# Autodesk Inventor assembly: Piston Build Platform assy
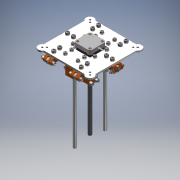
[picture p0: Inventor's stored thumbnail of the model, 180x180]
Saved by Autodesk Inventor 2018 (Build 220112000, 112)
## iProperties
Created: 2017-09-27
Part Number: Piston Build Platform assy
Document SubType Name: Assembly
Designer: Gabriel Smolnycki
Author: Gabriel Smolnycki
## Documents named in this file (11)
- H:\dev\planb\mechanics\V1INV\Subassemblies\Piston Build Platform assy.iam
- H:\dev\planb\mechanics\V1INV\Piston\Piston Build Frame.ipt
- H:\dev\planb\mechanics\V1INV\Subassemblies\Piston Wall Guide assy.iam
- H:\dev\planb\mechanics\V1INV\Hardware\M4 SS Washer.ipt
- H:\dev\planb\mechanics\V1INV\Hardware\M4 SS Locknut.ipt
- H:\dev\planb\mechanics\V1INV\Hardware\M4x25 SS SHCS.ipt
- H:\dev\planb\mechanics\V1INV\Subassemblies\Piston Motor Holder assy.iam
- H:\dev\planb\mechanics\V1INV\Hardware\M4x12 SS SHCS.ipt
- H:\dev\planb\mechanics\V1INV\Hardware\M4x30 SS Standoff FF (94868A183).ipt
- H:\dev\planb\mechanics\V1INV\Subassemblies\Piston Guide assy.iam
- H:\dev\planb\mechanics\V1INV\Hardware\M4x20 SS SHCS.ipt
## Components (118 placed, 10 different names)
1. Piston Build Frame:1 — Insert:1, Insert:2, Insert:3, Insert:4, Insert:5, Insert:6, Insert:7, Insert:8, Insert:9, Insert:10, Insert:11, Insert:12, Insert:13, Insert:14, Insert:15, Insert:16, Insert:17, Insert:18, Insert:19, Insert:20, Insert:21, Insert:22, Insert:23, Insert:24, Insert:61, Insert:62, Insert:63, Insert:64, Insert:65, Insert:66, Insert:67, Insert:68, Insert:91, Insert:92, Insert:93, Insert:94, Insert:95, Insert:96, Insert:97, Insert:98, Insert:99, Insert:100, Insert:101, Insert:102
2. Piston Wall Guide assy:1 [sub-assembly] — Insert:1, Insert:2, Insert:27, Insert:28
3. Piston Wall Guide assy:2 [sub-assembly] — Insert:3, Insert:4, Insert:25, Insert:26
4. Piston Wall Guide assy:3 [sub-assembly] — Insert:7, Insert:8, Insert:31, Insert:32
5. Piston Wall Guide assy:4 [sub-assembly] — Insert:5, Insert:6, Insert:29, Insert:30
6. Piston Wall Guide assy:5 [sub-assembly] — Insert:11, Insert:12, Insert:35, Insert:36
7. Piston Wall Guide assy:6 [sub-assembly] — Insert:9, Insert:10, Insert:33, Insert:34
8. M4x25 SS SHCS:1
9. M4x25 SS SHCS:2
10. M4x25 SS SHCS:3
11. M4x25 SS SHCS:4
12. M4x25 SS SHCS:5
13. M4x25 SS SHCS:6
14. M4x25 SS SHCS:7
15. M4x25 SS SHCS:8
16. M4x25 SS SHCS:9
17. M4x25 SS SHCS:10
18. M4x25 SS SHCS:11
19. M4x25 SS SHCS:12
20. M4 SS Washer:1 — Insert:14
21. M4 SS Washer:2 — Insert:16
22. M4 SS Washer:3 — Insert:21
23. M4 SS Washer:4 — Insert:22
24. M4 SS Washer:5 — Insert:13
25. M4 SS Washer:6 — Insert:17
26. M4 SS Washer:7 — Insert:20
27. M4 SS Washer:8 — Insert:36, Insert:48
28. M4 SS Washer:9 — Insert:15
29. M4 SS Washer:10 — Insert:18
30. M4 SS Washer:11 — Insert:19
31. M4 SS Washer:12 — Insert:23
32. M4 SS Washer:13 — Insert:32, Insert:44
33. M4 SS Washer:14 — Insert:31, Insert:43
34. M4 SS Washer:15 — Insert:30, Insert:39
35. M4 SS Washer:16 — Insert:29, Insert:40
36. M4 SS Washer:17 — Insert:35, Insert:47
37. M4 SS Washer:18 — Insert:34, Insert:46
38. M4 SS Washer:19 — Insert:33, Insert:45
39. M4 SS Washer:20 — Insert:28, Insert:42
40. M4 SS Washer:21 — Insert:24
41. M4 SS Washer:22 — Insert:27, Insert:41
42. M4 SS Washer:23 — Insert:26, Insert:38
43. M4 SS Washer:24 — Insert:25, Insert:37
44. M4 SS Locknut:1 — Insert:46
45. M4 SS Locknut:2 — Insert:45
46. M4 SS Locknut:3 — Insert:43
47. M4 SS Locknut:4 — Insert:41
48. M4 SS Locknut:5 — Insert:39
49. M4 SS Locknut:6 — Insert:37
50. M4 SS Locknut:7 — Insert:48
51. M4 SS Locknut:8 — Insert:47
52. M4 SS Locknut:9 — Insert:44
53. M4 SS Locknut:10 — Insert:42
54. M4 SS Locknut:11 — Insert:40
55. M4 SS Locknut:12 — Insert:38
56. Piston Motor Holder assy:1 [sub-assembly] — Insert:73, Insert:74, Insert:75, Insert:76, Insert:77, Insert:78, Insert:79, Insert:80
57. M4x12 SS SHCS:1
58. M4x12 SS SHCS:2
59. M4x12 SS SHCS:3
60. M4x12 SS SHCS:4
61. M4 SS Washer:25 — Insert:64
62. M4 SS Washer:26 — Insert:63
63. M4 SS Washer:27 — Insert:62
64. M4 SS Washer:28 — Insert:61
65. M4 SS Washer:29 — Insert:66, Insert:86
66. M4 SS Washer:30 — Insert:67, Insert:85
67. M4 SS Washer:31 — Insert:68, Insert:87
68. M4 SS Washer:32 — Insert:65, Insert:88
69. M4 SS Washer:33 — Insert:73, Insert:84
70. M4 SS Washer:34 — Insert:80, Insert:90
71. M4 SS Washer:35 — Insert:79
72. M4 SS Washer:36 — Insert:78, Insert:89
73. M4 SS Washer:37 — Insert:74, Insert:83
74. M4 SS Washer:38 — Insert:75, Insert:81
75. M4 SS Washer:39 — Insert:76, Insert:82
76. M4 SS Washer:40 — Insert:77
77. M4x12 SS SHCS:5 — Insert:81
78. M4x12 SS SHCS:6 — Insert:82
79. M4x12 SS SHCS:7 — Insert:84
80. M4x12 SS SHCS:8 — Insert:83
81. M4x30 SS Standoff FF (94868A183):1 — Insert:85, Insert:89
82. M4x30 SS Standoff FF (94868A183):2 — Insert:86
83. M4x30 SS Standoff FF (94868A183):3 — Insert:87
84. M4x30 SS Standoff FF (94868A183):4 — Insert:88, Insert:90
85. Piston Guide assy:1 [sub-assembly] — Insert:91, Insert:92, Insert:107, Insert:108, Insert:109, Insert:110
86. Piston Guide assy:2 [sub-assembly] — Insert:93, Insert:94, Insert:103, Insert:104, Insert:105, Insert:106
87. M4x20 SS SHCS:1
88. M4x20 SS SHCS:2
89. M4x20 SS SHCS:3
90. M4x20 SS SHCS:4
91. M4x20 SS SHCS:5
92. M4x20 SS SHCS:6
93. M4x20 SS SHCS:7
94. M4x20 SS SHCS:8
95. M4 SS Washer:41 — Insert:95
96. M4 SS Washer:42 — Insert:96
97. M4 SS Washer:43 — Insert:97
98. M4 SS Washer:44 — Insert:98
99. M4 SS Washer:45 — Insert:99
100. M4 SS Washer:46 — Insert:100
101. M4 SS Washer:47 — Insert:101
102. M4 SS Washer:48 — Insert:102
103. M4 SS Washer:49 — Insert:106, Insert:118
104. M4 SS Washer:50 — Insert:107, Insert:114
105. M4 SS Washer:51 — Insert:108, Insert:111
106. M4 SS Washer:52 — Insert:109, Insert:112
107. M4 SS Washer:53 — Insert:103, Insert:116
108. M4 SS Washer:54 — Insert:104, Insert:115
109. M4 SS Washer:55 — Insert:105, Insert:117
110. M4 SS Washer:56 — Insert:110, Insert:113
111. M4 SS Locknut:13 — Insert:111
112. M4 SS Locknut:14 — Insert:112
113. M4 SS Locknut:15 — Insert:113
114. M4 SS Locknut:16 — Insert:114
115. M4 SS Locknut:17 — Insert:115
116. M4 SS Locknut:18 — Insert:116
117. M4 SS Locknut:19 — Insert:117
118. M4 SS Locknut:20 — Insert:118
## Relationships (126: Insert 126)
- Insert:1: Piston Build Frame:1 ↔ Piston Wall Guide assy:1
- Insert:2: Piston Build Frame:1 ↔ Piston Wall Guide assy:1
- Insert:3: Piston Build Frame:1 ↔ Piston Wall Guide assy:2
- Insert:4: Piston Build Frame:1 ↔ Piston Wall Guide assy:2
- Insert:5: Piston Build Frame:1 ↔ Piston Wall Guide assy:4
- Insert:6: Piston Build Frame:1 ↔ Piston Wall Guide assy:4
- Insert:7: Piston Build Frame:1 ↔ Piston Wall Guide assy:3
- Insert:8: Piston Build Frame:1 ↔ Piston Wall Guide assy:3
- Insert:9: Piston Build Frame:1 ↔ Piston Wall Guide assy:6
- Insert:10: Piston Build Frame:1 ↔ Piston Wall Guide assy:6
- Insert:11: Piston Build Frame:1 ↔ Piston Wall Guide assy:5
- Insert:12: Piston Build Frame:1 ↔ Piston Wall Guide assy:5
- Insert:13: Piston Build Frame:1 ↔ M4 SS Washer:5
- Insert:14: Piston Build Frame:1 ↔ M4 SS Washer:1
- Insert:15: Piston Build Frame:1 ↔ M4 SS Washer:9
- Insert:16: Piston Build Frame:1 ↔ M4 SS Washer:2
- Insert:17: Piston Build Frame:1 ↔ M4 SS Washer:6
- Insert:18: Piston Build Frame:1 ↔ M4 SS Washer:10
- Insert:19: Piston Build Frame:1 ↔ M4 SS Washer:11
- Insert:20: Piston Build Frame:1 ↔ M4 SS Washer:7
- Insert:21: Piston Build Frame:1 ↔ M4 SS Washer:3
- Insert:22: Piston Build Frame:1 ↔ M4 SS Washer:4
- Insert:23: Piston Build Frame:1 ↔ M4 SS Washer:12
- Insert:24: Piston Build Frame:1 ↔ M4 SS Washer:21
- Insert:25: Piston Wall Guide assy:2 ↔ M4 SS Washer:24
- Insert:26: Piston Wall Guide assy:2 ↔ M4 SS Washer:23
- Insert:27: Piston Wall Guide assy:1 ↔ M4 SS Washer:22
- Insert:28: Piston Wall Guide assy:1 ↔ M4 SS Washer:20
- Insert:29: Piston Wall Guide assy:4 ↔ M4 SS Washer:16
- Insert:30: Piston Wall Guide assy:4 ↔ M4 SS Washer:15
- Insert:31: Piston Wall Guide assy:3 ↔ M4 SS Washer:14
- Insert:32: Piston Wall Guide assy:3 ↔ M4 SS Washer:13
- Insert:33: Piston Wall Guide assy:6 ↔ M4 SS Washer:19
- Insert:34: Piston Wall Guide assy:6 ↔ M4 SS Washer:18
- Insert:35: Piston Wall Guide assy:5 ↔ M4 SS Washer:17
- Insert:36: Piston Wall Guide assy:5 ↔ M4 SS Washer:8
- Insert:37: M4 SS Washer:24 ↔ M4 SS Locknut:6
- Insert:38: M4 SS Washer:23 ↔ M4 SS Locknut:12
- Insert:39: M4 SS Washer:15 ↔ M4 SS Locknut:5
- Insert:40: M4 SS Washer:16 ↔ M4 SS Locknut:11
- Insert:41: M4 SS Washer:22 ↔ M4 SS Locknut:4
- Insert:42: M4 SS Washer:20 ↔ M4 SS Locknut:10
- Insert:43: M4 SS Washer:14 ↔ M4 SS Locknut:3
- Insert:44: M4 SS Washer:13 ↔ M4 SS Locknut:9
- Insert:45: M4 SS Washer:19 ↔ M4 SS Locknut:2
- Insert:46: M4 SS Washer:18 ↔ M4 SS Locknut:1
- Insert:47: M4 SS Washer:17 ↔ M4 SS Locknut:8
- Insert:48: M4 SS Washer:8 ↔ M4 SS Locknut:7
- [Insert]: M4x25 SS SHCS:12 ↔ M4 SS Washer:9
- [Insert]: M4x25 SS SHCS:11 ↔ M4 SS Washer:2
- [Insert]: M4x25 SS SHCS:3 ↔ M4 SS Washer:6
- [Insert]: M4x25 SS SHCS:4 ↔ M4 SS Washer:10
- [Insert]: M4x25 SS SHCS:5 ↔ M4 SS Washer:7
- [Insert]: M4x25 SS SHCS:6 ↔ M4 SS Washer:11
- [Insert]: M4x25 SS SHCS:9 ↔ M4 SS Washer:5
- [Insert]: M4x25 SS SHCS:10 ↔ M4 SS Washer:1
- [Insert]: M4x25 SS SHCS:1 ↔ M4 SS Washer:12
- [Insert]: M4x25 SS SHCS:2 ↔ M4 SS Washer:21
- [Insert]: M4x25 SS SHCS:7 ↔ M4 SS Washer:3
- [Insert]: M4x25 SS SHCS:8 ↔ M4 SS Washer:4
- Insert:61: Piston Build Frame:1 ↔ M4 SS Washer:28
- Insert:62: Piston Build Frame:1 ↔ M4 SS Washer:27
- Insert:63: Piston Build Frame:1 ↔ M4 SS Washer:26
- Insert:64: Piston Build Frame:1 ↔ M4 SS Washer:25
- Insert:65: Piston Build Frame:1 ↔ M4 SS Washer:32
- Insert:66: Piston Build Frame:1 ↔ M4 SS Washer:29
- Insert:67: Piston Build Frame:1 ↔ M4 SS Washer:30
- Insert:68: Piston Build Frame:1 ↔ M4 SS Washer:31
- [Insert]: M4x12 SS SHCS:1 ↔ M4 SS Washer:27
- [Insert]: M4x12 SS SHCS:3 ↔ M4 SS Washer:28
- [Insert]: M4x12 SS SHCS:2 ↔ M4 SS Washer:25
- [Insert]: M4x12 SS SHCS:4 ↔ M4 SS Washer:26
- Insert:73: Piston Motor Holder assy:1 ↔ M4 SS Washer:33
- Insert:74: Piston Motor Holder assy:1 ↔ M4 SS Washer:37
- Insert:75: Piston Motor Holder assy:1 ↔ M4 SS Washer:38
- Insert:76: Piston Motor Holder assy:1 ↔ M4 SS Washer:39
- Insert:77: Piston Motor Holder assy:1 ↔ M4 SS Washer:40
- Insert:78: Piston Motor Holder assy:1 ↔ M4 SS Washer:36
- Insert:79: Piston Motor Holder assy:1 ↔ M4 SS Washer:35
- Insert:80: Piston Motor Holder assy:1 ↔ M4 SS Washer:34
- Insert:81: M4 SS Washer:38 ↔ M4x12 SS SHCS:5
- Insert:82: M4 SS Washer:39 ↔ M4x12 SS SHCS:6
- Insert:83: M4 SS Washer:37 ↔ M4x12 SS SHCS:8
- Insert:84: M4 SS Washer:33 ↔ M4x12 SS SHCS:7
- Insert:85: M4 SS Washer:30 ↔ M4x30 SS Standoff FF (94868A183):1
- Insert:86: M4 SS Washer:29 ↔ M4x30 SS Standoff FF (94868A183):2
- Insert:87: M4 SS Washer:31 ↔ M4x30 SS Standoff FF (94868A183):3
- Insert:88: M4 SS Washer:32 ↔ M4x30 SS Standoff FF (94868A183):4
- Insert:89: M4 SS Washer:36 ↔ M4x30 SS Standoff FF (94868A183):1
- Insert:90: M4 SS Washer:34 ↔ M4x30 SS Standoff FF (94868A183):4
- Insert:91: Piston Build Frame:1 ↔ Piston Guide assy:1
- Insert:92: Piston Build Frame:1 ↔ Piston Guide assy:1
- Insert:93: Piston Build Frame:1 ↔ Piston Guide assy:2
- Insert:94: Piston Build Frame:1 ↔ Piston Guide assy:2
- Insert:95: Piston Build Frame:1 ↔ M4 SS Washer:41
- Insert:96: Piston Build Frame:1 ↔ M4 SS Washer:42
- Insert:97: Piston Build Frame:1 ↔ M4 SS Washer:43
- Insert:98: Piston Build Frame:1 ↔ M4 SS Washer:44
- Insert:99: Piston Build Frame:1 ↔ M4 SS Washer:45
- Insert:100: Piston Build Frame:1 ↔ M4 SS Washer:46
- Insert:101: Piston Build Frame:1 ↔ M4 SS Washer:47
- Insert:102: Piston Build Frame:1 ↔ M4 SS Washer:48
- Insert:103: Piston Guide assy:2 ↔ M4 SS Washer:53
- Insert:104: Piston Guide assy:2 ↔ M4 SS Washer:54
- Insert:105: Piston Guide assy:2 ↔ M4 SS Washer:55
- Insert:106: Piston Guide assy:2 ↔ M4 SS Washer:49
- Insert:107: Piston Guide assy:1 ↔ M4 SS Washer:50
- Insert:108: Piston Guide assy:1 ↔ M4 SS Washer:51
- Insert:109: Piston Guide assy:1 ↔ M4 SS Washer:52
- Insert:110: Piston Guide assy:1 ↔ M4 SS Washer:56
- Insert:111: M4 SS Washer:51 ↔ M4 SS Locknut:13
- Insert:112: M4 SS Washer:52 ↔ M4 SS Locknut:14
- Insert:113: M4 SS Washer:56 ↔ M4 SS Locknut:15
- Insert:114: M4 SS Washer:50 ↔ M4 SS Locknut:16
- Insert:115: M4 SS Washer:54 ↔ M4 SS Locknut:17
- Insert:116: M4 SS Washer:53 ↔ M4 SS Locknut:18
- Insert:117: M4 SS Washer:55 ↔ M4 SS Locknut:19
- Insert:118: M4 SS Washer:49 ↔ M4 SS Locknut:20
- [Insert]: M4x20 SS SHCS:1 ↔ M4 SS Washer:41
- [Insert]: M4x20 SS SHCS:2 ↔ M4 SS Washer:42
- [Insert]: M4x20 SS SHCS:3 ↔ M4 SS Washer:43
- [Insert]: M4x20 SS SHCS:4 ↔ M4 SS Washer:44
- [Insert]: M4x20 SS SHCS:5 ↔ M4 SS Washer:45
- [Insert]: M4x20 SS SHCS:6 ↔ M4 SS Washer:46
- [Insert]: M4x20 SS SHCS:7 ↔ M4 SS Washer:47
- [Insert]: M4x20 SS SHCS:8 ↔ M4 SS Washer:48
